# Autodesk Inventor assembly: Assembly1
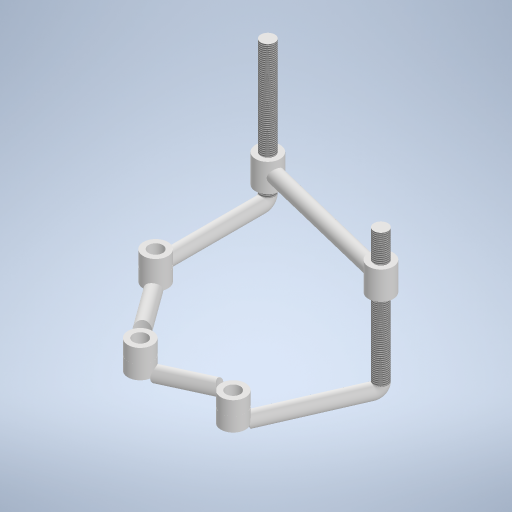
[picture p0: Inventor's stored thumbnail of the model, 512x512]
Saved by Autodesk Inventor 2024 (Build 280153000, 153)
## iProperties
Created: 2023-10-11
Part Number: Assembly1
Document SubType Name: Assembly
Designer: owner
Author: owner
## Documents named in this file (4)
- C:\Users\owner\Documents\institute_information\高等機動學\hw1\Assembly1.iam
- C:\Users\owner\Documents\institute_information\高等機動學\hw1\Part1.ipt
- C:\Users\owner\Documents\institute_information\高等機動學\hw1\Part3.ipt
- C:\Users\owner\Documents\institute_information\高等機動學\hw1\Part4.ipt
## Components (5 placed, 3 different names)
1. Part1:1 — Mate:7, Flush:1, Mate:13, Mate:16
2. Part1:2 — Mate:8, Mate:10, Mate:12
3. Part4:1 — Mate:7, Mate:8, Flush:1
4. Part3:1 — Mate:10, Mate:12, Mate:14, Mate:15
5. Part3:2 — Mate:13, Mate:14, Mate:15, Mate:16
## Relationships (9: Mate 8, Flush 1)
- Mate:7: Part1:1 ↔ Part4:1
- Mate:8: Part1:2 ↔ Part4:1
- Mate:10: Part1:2 ↔ Part3:1
- Mate:12: Part1:2 ↔ Part3:1
- Flush:1 (-140 mm): Part1:1 ↔ Part4:1
- Mate:13: Part1:1 ↔ Part3:2
- Mate:14: Part3:1 ↔ Part3:2
- Mate:15: Part3:1 ↔ Part3:2
- Mate:16: Part1:1 ↔ Part3:2
